# Autodesk Inventor assembly: 739276
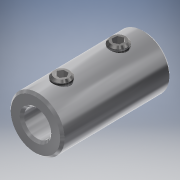
[picture p0: Inventor's stored thumbnail of the model, 180x180]
Saved by Autodesk Inventor 2019 (Build 230136000, 136)
## iProperties
Category: Fasteners
Company: Autodesk Inc.
Created: 2014-11-27
Part Number: 739276
Document SubType Name: Assembly
Designer: Tetrix
Catalog Web Link: http://www.tetrixrobotics.com/TETRIX_Motor-Axle_Shaft_Couplers
Vendor: Tetrix
Mass: 6.68388 g
Surface Area: 17.5666 cm^2
Volume: 2.2843 cm^3
Density: 2.926 g/cm^3
Author: Autodesk Inc.
## Documents named in this file (3)
- C:\Users\tbloo\Documents\Inventor\FTC Tetrix KOP\Miscellaneous\Tetrix_39276.iam
- C:\Users\tbloo\Downloads\FTC Tetrix KOP\Miscellaneous\Tetrix_39276_Body.ipt
- C:\Users\tbloo\Downloads\FTC Tetrix KOP\Miscellaneous\Tetrix_39276_Screw.ipt
## Components (3 placed, 2 different names)
1. Tetrix_39276_Body:1 — Mate:1, Mate:2
2. Tetrix_739275_Screw:1 — Mate:1, Flush:1
3. Tetrix_739275_Screw:2 — Mate:2, Flush:1
## Relationships (3: Mate 2, Flush 1)
- Mate:1: Tetrix_39276_Body:1 ↔ Tetrix_739275_Screw:1
- Mate:2: Tetrix_39276_Body:1 ↔ Tetrix_739275_Screw:2
- Flush:1: Tetrix_739275_Screw:1 ↔ Tetrix_739275_Screw:2
